# Autodesk Inventor assembly: BarBot_Frame
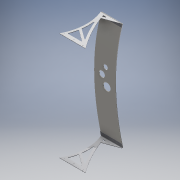
[picture p0: Inventor's stored thumbnail of the model, 180x180]
Saved by Autodesk Inventor 2016 (Build 200138000, 138)
## iProperties
Created: 2016-04-15
Part Number: BarBot_Frame
Document SubType Name: Assembly
Designer: 3DPrinterUser
Author: 3DPrinterUser
## Documents named in this file (7)
- X:\Projekte Bastli\BarBot\Conception\Mechanical\BarBot_Frame\BarBot_Frame.iam
- X:\Projekte Bastli\BarBot\Conception\Mechanical\BarBot_Frame\Floor.ipt
- X:\Projekte Bastli\BarBot\Conception\Mechanical\BarBot_Frame\Foot_left.ipt
- X:\Projekte Bastli\BarBot\Conception\Mechanical\BarBot_Frame\Foot_Right.ipt
- X:\Projekte Bastli\BarBot\Conception\Mechanical\BarBot_Frame\Side_Fixture.ipt
- X:\Projekte Bastli\BarBot\Conception\Mechanical\BarBot_Frame\Side_Fixture_Mirrored.ipt
- X:\Projekte Bastli\BarBot\Conception\Mechanical\BarBot_Frame\Top_Blade.ipt
## Components (6 placed, 6 different names)
1. Floor:1 — Flush:1, Flush:2, Flush:3, Rigid:1
2. Foot_left:1 — Flush:1, Flush:2, Flush:3, Flush:4, Flush:5
3. Foot_Right:1 — Rigid:1, Rigid:2
4. Side_Fixture:1 — Flush:4, Flush:5, Flush:6, Flush:7
5. Side_Fixture_Mirrored:1 — Rigid:2
6. Top_Blade:1 — Flush:6, Flush:7
## Relationships (9: Flush 7, WeldJoint 2)
- Flush:1: Floor:1 ↔ Foot_left:1
- Flush:2: Floor:1 ↔ Foot_left:1
- Flush:3: Floor:1 ↔ Foot_left:1
- Rigid:1 [WeldJoint]: Floor:1 ↔ Foot_Right:1
- Flush:4: Foot_left:1 ↔ Side_Fixture:1
- Flush:5: Foot_left:1 ↔ Side_Fixture:1
- Rigid:2 [WeldJoint]: Foot_Right:1 ↔ Side_Fixture_Mirrored:1
- Flush:6: Side_Fixture:1 ↔ Top_Blade:1
- Flush:7: Side_Fixture:1 ↔ Top_Blade:1
